# Autodesk Inventor assembly: nieuwe voetensteun
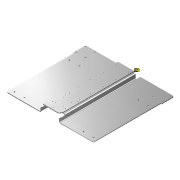
[picture p0: Inventor's stored thumbnail of the model, 180x180]
Saved by Autodesk Inventor 2020.3 (Build 243373000, 373)
## iProperties
Created: 2020-12-09
Part Number: nieuwe voetensteun
Document SubType Name: Assembly
Designer: Svend
Author: Svend
## Documents named in this file (3)
- C:\Users\Svend\OneDrive\Documents\GitHub\Rolstoel\nieuwe voetensteun.iam
- C:\Users\Svend\OneDrive\Documents\GitHub\Rolstoel\voetensteun middenstuk.ipt
- C:\Users\Svend\OneDrive\Documents\GitHub\Rolstoel\voetensteun zijkanten.ipt
## Components (2 placed, 2 different names)
1. voetensteun middenstuk:1 — Mate:1, Flush:2, Mate:2
2. voetensteun zijkanten:1 — Mate:1, Flush:2, Mate:2
## Relationships (3: Mate 2, Flush 1)
- Mate:1: voetensteun middenstuk:1 ↔ voetensteun zijkanten:1
- Flush:2: voetensteun middenstuk:1 ↔ voetensteun zijkanten:1
- Mate:2 (-20 mm): voetensteun middenstuk:1 ↔ voetensteun zijkanten:1
